# Autodesk Inventor assembly: bearing_fc12025_s09_cross_section
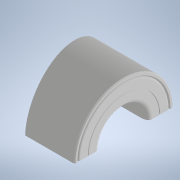
[picture p0: Inventor's stored thumbnail of the model, 180x180]
Saved by Autodesk Inventor 2021.1 (Build 251245010, 245A)
## iProperties
Created: 2025-07-24
Part Number: bearing_fc12025_s09_cross_section
Document SubType Name: Assembly
Designer: Anton.Birukov
Sending System: CREO PARAMETRIC BY PTC INC, 2024374
Preprocessor: CREO PARAMETRIC BY PTC INC, 2024374
Title: BEARING_FC12025_S09_ASM
Author: User
Revision Number: 4LAST_VERSION
## Documents named in this file (7)
- D:\Работа\DTscan\Анализ подшипников\Запись данных на стенде\Bearing_testing\bearing_fc12025_s09_cross_section.iam
- D:\Работа\DTscan\Анализ подшипников\Запись данных на стенде\Bearing_testing\OUTER_RING.ipt
- D:\Работа\DTscan\Анализ подшипников\Запись данных на стенде\Bearing_testing\INNER_RING.ipt
- D:\Работа\DTscan\Анализ подшипников\Запись данных на стенде\Bearing_testing\SEPARATOR.ipt
- D:\Работа\DTscan\Анализ подшипников\Запись данных на стенде\Bearing_testing\SEAL.ipt
- D:\Работа\DTscan\Анализ подшипников\Запись данных на стенде\Bearing_testing\ROLL.ipt
- D:\Работа\DTscan\Анализ подшипников\Запись данных на стенде\Bearing_testing\BRACKET.ipt
## Components (42 placed, 42 different names)
1. 0
2. 1 — Совмещение:1, Совмещение:2
3. 2
4. 3
5. 4
6. 5
7. 6
8. 7
9. 8
10. 9
11. 10
12. 11
13. 12
14. 13 — Заподлицо:1
15. 14
16. 15
17. 16
18. 17
19. 18
20. 19
21. 20
22. 21
23. 22
24. 23
25. 24
26. 25
27. 26
28. 27
29. 28
30. 29
31. 30
32. 31
33. 32
34. 33
35. 34
36. 35
37. 36
38. 37
39. 38
40. 39
41. 40
42. 41
## Relationships (4: Mate 3, Flush 1)
- Заподлицо:1 [Flush] (-5.4 mm): 13
- Совмещение:1 [Mate]: 1
- Совмещение:2 [Mate]: 1
- Совмещение:3 [Mate]
